# Autodesk Inventor assembly: 2018 Build Model
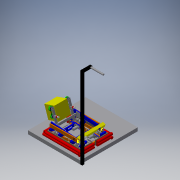
[picture p0: Inventor's stored thumbnail of the model, 180x180]
Saved by Autodesk Inventor 2018 (Build 220112000, 112)
## iProperties
Created: 2016-01-11
Part Number: 2018 Build Model
Document SubType Name: Assembly
Designer: Applegate
Author: Applegate
## Documents named in this file (6)
- C:\Users\Apple\Documents\Inventor\2018 PowerUp\2018 Platform Zone w robot.iam
- C:\Users\Apple\Documents\Inventor\2018 PowerUp\Ramp.ipt
- C:\Users\Apple\Documents\Inventor\2018 PowerUp\Vertical Rung.ipt
- C:\Users\Apple\Documents\Inventor\2018 PowerUp\Rung Support.ipt
- C:\Users\Apple\Documents\Inventor\2018 PowerUp\Rung Bar.ipt
- C:\Users\Apple\Documents\Inventor\2018 PowerUp\2018 Robot.iam
## Components (5 placed, 5 different names)
1. Ramp:1 — Flush:1, Flush:4, Mate:4, Flush:5, Mate:10, Flush:11
2. Vertical Rung:1 — Flush:4, Mate:4, Flush:5, Flush:7, Mate:7, Flush:10, Mate:11
3. Rung Support:1 — Flush:7, Flush:9, Mate:6, Mate:7, Flush:10
4. Rung Bar:1 — Flush:9, Mate:6
5. 2018 Robot:1 [sub-assembly] — Mate:10, Mate:11, Flush:11
## Relationships (12: Flush 7, Mate 5)
- Flush:1: Ramp:1
- Flush:4: Ramp:1 ↔ Vertical Rung:1
- Mate:4: Ramp:1 ↔ Vertical Rung:1
- Flush:5: Ramp:1 ↔ Vertical Rung:1
- Flush:7: Vertical Rung:1 ↔ Rung Support:1
- Flush:9: Rung Support:1 ↔ Rung Bar:1
- Mate:6: Rung Support:1 ↔ Rung Bar:1
- Mate:7: Vertical Rung:1 ↔ Rung Support:1
- Flush:10: Vertical Rung:1 ↔ Rung Support:1
- Mate:10 (63.5 mm): Ramp:1 ↔ 2018 Robot:1
- Mate:11: Vertical Rung:1 ↔ 2018 Robot:1
- Flush:11: Ramp:1 ↔ 2018 Robot:1
